# Autodesk Inventor assembly: JewlArm
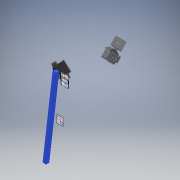
[picture p0: Inventor's stored thumbnail of the model, 180x180]
Saved by Autodesk Inventor 2017 (Build 210142000, 142)
## iProperties
Created: 2017-10-12
Part Number: JewlArm
Document SubType Name: Assembly
Designer: User
Author: User
## Documents named in this file (5)
- C:\Robotics\CAD\2017-18_CAD\JewlArm.iam
- C:\Robotics\CAD\COTSParts\Tetrix\Tetrix servo 180.ipt
- C:\Robotics\CAD\COTSParts\Tetrix\Tetrix bracket - single servo.ipt
- C:\Robotics\CAD\COTSParts\Tetrix\Tetrix channel 32mm.ipt
- C:\Robotics\CAD\2017-18_CAD\jewlArmBeam.ipt
## Components (6 placed, 4 different names)
1. Tetrix servo 180:1 — Insert:5, Insert:7, Mate:3, Mate:4
2. Tetrix servo 180:2 — Mate:11, Mate:12, Mate:14, Mate:15, Mate:16, Mate:17
3. Tetrix bracket - single servo:1 — Mate:11, Mate:12
4. Tetrix bracket - single servo:2 — Insert:5, Mate:3
5. Tetrix channel 32mm:1 — Insert:7, Mate:4
6. jewlArmBeam:1 — Mate:14, Mate:15, Mate:16, Mate:17
## Relationships (10: Mate 8, Insert 2)
- Insert:5: Tetrix servo 180:1 ↔ Tetrix bracket - single servo:2
- Insert:7: Tetrix servo 180:1 ↔ Tetrix channel 32mm:1
- Mate:11: Tetrix servo 180:2 ↔ Tetrix bracket - single servo:1
- Mate:3: Tetrix servo 180:1 ↔ Tetrix bracket - single servo:2
- Mate:4: Tetrix servo 180:1 ↔ Tetrix channel 32mm:1
- Mate:12: Tetrix servo 180:2 ↔ Tetrix bracket - single servo:1
- Mate:14: Tetrix servo 180:2 ↔ jewlArmBeam:1
- Mate:15: Tetrix servo 180:2 ↔ jewlArmBeam:1
- Mate:16 (0.254 mm): Tetrix servo 180:2 ↔ jewlArmBeam:1
- Mate:17: Tetrix servo 180:2 ↔ jewlArmBeam:1
